# Autodesk Inventor assembly: Сервопривод с кареткой
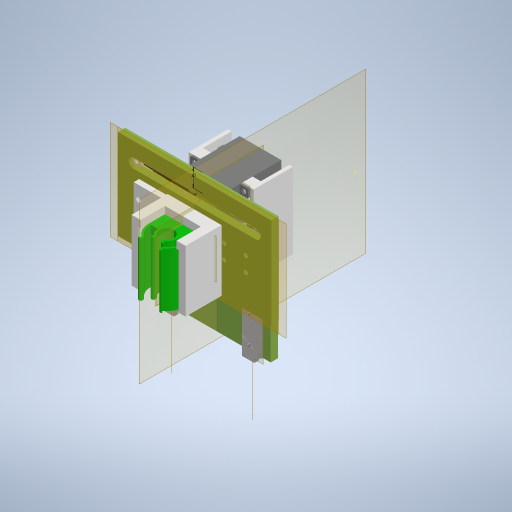
[picture p0: Inventor's stored thumbnail of the model, 512x512]
Saved by Autodesk Inventor 2024.2 (Build 282272000, 272)
## iProperties
Created: 2025-11-27
Part Number: Сервопривод с кареткой
Document SubType Name: Assembly
Designer: katya_notebook
Author: katya_notebook
## Documents named in this file (15)
- E:\ETZ_9\construction\Сервопривод с кареткой.iam
- E:\ETZ_9\construction\JX Servo PDI-HV2006MG\JX Servo PDI-HV2006MG.ipt
- E:\ETZ_9\construction\MGN7C каретка\MGN7C каретка.ipt
- E:\ETZ_9\construction\MHN7C рельса\MHN7C рельса.ipt
- E:\ETZ_9\construction\крепление рельс.ipt
- E:\ETZ_9\construction\крепление каретки.ipt
- E:\ETZ_9\construction\подшипник мини.ipt
- E:\ETZ_9\construction\деталь которая двигает.ipt
- E:\ETZ_9\construction\деталь на которой рельсы.ipt
- E:\ETZ_9\construction\25T Servo Horn Steering Arm M3 версия 3.ipt
- E:\ETZ_9\construction\держатель сервомоторчика.ipt
- E:\ETZ_9\construction\крепление маркера 8мм.ipt
- E:\ETZ_9\construction\печать\держатель магнитов на основе.ipt
- E:\ETZ_9\construction\крепление маркера 18мм.ipt
- E:\ETZ_9\construction\печать\проставк.ipt
## Components (16 placed, 14 different names)
1. JX Servo PDI-HV2006MG:1 — Совмещение:5, Совмещение:9, Совмещение:10, С поворотом:1, Совмещение:11, Заподлицо:5
2. MGN7C каретка:1 — Жесткий:2, Совмещение:8
3. MHN7C рельса:1 — Совмещение:2, Заподлицо:1, Совмещение:3, Совмещение:4, Жесткий:2, Совмещение:6, Совмещение:7, Заподлицо:3
4. крепление рельс:1
5. крепление каретки:1
6. подшипник мини:1 — Совмещение:12
7. MHN7C рельса:2 — Заподлицо:1, Совмещение:3, Совмещение:6, Совмещение:7, Жесткий:3
8. MGN7C каретка:2 — Жесткий:3, Совмещение:8, Заподлицо:4, Совмещение:11
9. деталь которая двигает:1 — Заподлицо:3
10. деталь на которой рельсы:1 — Заподлицо:4, Совмещение:9, Заподлицо:6, Заподлицо:8, Заподлицо:9, Заподлицо:10
11. 25T Servo Horn Steering Arm M3 версия 3:1 — Совмещение:10, С поворотом:1, Совмещение:12
12. держатель сервомоторчика:1 — Заподлицо:5
13. крепление маркера 8мм:1 — Заподлицо:6, Заподлицо:7
14. держатель магнитов на основе:1 — Заподлицо:8, Заподлицо:9, Заподлицо:10
15. крепление маркера 18мм:1
16. проставк:1
## Relationships (23: Mate 11, Flush 9, WeldJoint 2, RevoluteJoint 1)
- Совмещение:2 [Mate]: MHN7C рельса:1
- Заподлицо:1 [Flush]: MHN7C рельса:1 ↔ MHN7C рельса:2
- Совмещение:3 [Mate] (38 mm): MHN7C рельса:1 ↔ MHN7C рельса:2
- Совмещение:4 [Mate] (22.3 mm): MHN7C рельса:1
- Совмещение:5 [Mate]: JX Servo PDI-HV2006MG:1
- Жесткий:2 [WeldJoint]: MGN7C каретка:1 ↔ MHN7C рельса:1
- Совмещение:6 [Mate]: MHN7C рельса:1 ↔ MHN7C рельса:2
- Совмещение:7 [Mate]: MHN7C рельса:1 ↔ MHN7C рельса:2
- Жесткий:3 [WeldJoint]: MHN7C рельса:2 ↔ MGN7C каретка:2
- Совмещение:8 [Mate]: MGN7C каретка:1 ↔ MGN7C каретка:2
- Заподлицо:3 [Flush]: MHN7C рельса:1 ↔ деталь которая двигает:1
- Заподлицо:4 [Flush]: MGN7C каретка:2 ↔ деталь на которой рельсы:1
- Совмещение:9 [Mate] (4.5 mm): JX Servo PDI-HV2006MG:1 ↔ деталь на которой рельсы:1
- Совмещение:10 [Mate]: JX Servo PDI-HV2006MG:1 ↔ 25T Servo Horn Steering Arm M3 версия 3:1
- С поворотом:1 [RevoluteJoint]: JX Servo PDI-HV2006MG:1 ↔ 25T Servo Horn Steering Arm M3 версия 3:1
- Совмещение:11 [Mate]: JX Servo PDI-HV2006MG:1 ↔ MGN7C каретка:2
- Совмещение:12 [Mate]: подшипник мини:1 ↔ 25T Servo Horn Steering Arm M3 версия 3:1
- Заподлицо:5 [Flush]: JX Servo PDI-HV2006MG:1 ↔ держатель сервомоторчика:1
- Заподлицо:6 [Flush]: деталь на которой рельсы:1 ↔ крепление маркера 8мм:1
- Заподлицо:7 [Flush]: крепление маркера 8мм:1
- Заподлицо:8 [Flush]: деталь на которой рельсы:1 ↔ держатель магнитов на основе:1
- Заподлицо:9 [Flush] (-27.55 mm): деталь на которой рельсы:1 ↔ держатель магнитов на основе:1
- Заподлицо:10 [Flush]: деталь на которой рельсы:1 ↔ держатель магнитов на основе:1
